# Autodesk Inventor assembly: assembly_support
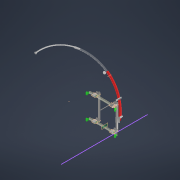
[picture p0: Inventor's stored thumbnail of the model, 180x180]
Saved by Autodesk Inventor 2021 (Build 250183000, 183)
## iProperties
Created: 2021-05-11
Part Number: assembly_support
Document SubType Name: Assembly
Designer: Watchdog
Author: Watchdog
## Documents named in this file (6)
- C:\Users\Watchdog\OneDrive - Flinders\Advn Mech Design Shared\6_Development\2_Design\inventor\support\assembly_support.iam
- C:\Users\Watchdog\OneDrive - Flinders\Advn Mech Design Shared\6_Development\2_Design\inventor\support\roof_bar\ext_roof bar assembly.iam
- C:\Users\Watchdog\OneDrive - Flinders\Advn Mech Design Shared\6_Development\2_Design\inventor\connection\assembly_connector.iam
- C:\Users\Watchdog\OneDrive - Flinders\Advn Mech Design Shared\6_Development\2_Design\inventor\assembly_hoop.iam
- C:\Users\Watchdog\OneDrive - Flinders\Advn Mech Design Shared\6_Development\2_Design\inventor\support\assembly_truss.iam
- C:\Users\Watchdog\OneDrive - Flinders\Advn Mech Design Shared\6_Development\2_Design\inventor\support\support_frame_x.ipt
## Components (9 placed, 5 different names)
1. ext_roof bar assembly:1 [sub-assembly] — Flush:6, Flush:7, Flush:8, Mate:15, Mate:16, Mate:18, Mate:20
2. ext_roof bar assembly:2 [sub-assembly] — Flush:3, Flush:4, Flush:5, Flush:6, Flush:7, Flush:8, Flush:9, Mate:11, Mate:13, Mate:14
3. assembly_connector:1 [sub-assembly] — Flush:9, Mate:11, Mate:21
4. assembly_connector:2 [sub-assembly] — Mate:13, Mate:14, Flush:11, Mate:27
5. assembly_connector:3 [sub-assembly] — Mate:15, Mate:16, Flush:10, Flush:11, Symmetry:1, Mate:26, Mate:28
6. assembly_connector:4 [sub-assembly] — Mate:18, Mate:20, Mate:22, Mate:23, Flush:10, Symmetry:1
7. assembly_hoop:1 [sub-assembly] — Mate:21, Mate:22, Mate:23, Mate:24, Mate:29, Flush:12
8. assembly_truss:1 [sub-assembly] — Mate:24, Mate:29, Flush:12
9. support_frame_x:1 — Mate:26, Mate:27, Mate:28
## Relationships (26: Mate 15, Flush 10, Symmetry 1)
- Flush:3: ext_roof bar assembly:2
- Flush:4: ext_roof bar assembly:2
- Flush:5: ext_roof bar assembly:2
- Flush:6 (900 mm): ext_roof bar assembly:1 ↔ ext_roof bar assembly:2
- Flush:7: ext_roof bar assembly:1 ↔ ext_roof bar assembly:2
- Flush:8: ext_roof bar assembly:1 ↔ ext_roof bar assembly:2
- Flush:9: ext_roof bar assembly:2 ↔ assembly_connector:1
- Mate:11: ext_roof bar assembly:2 ↔ assembly_connector:1
- Mate:13: ext_roof bar assembly:2 ↔ assembly_connector:2
- Mate:14: ext_roof bar assembly:2 ↔ assembly_connector:2
- Mate:15: ext_roof bar assembly:1 ↔ assembly_connector:3
- Mate:16: ext_roof bar assembly:1 ↔ assembly_connector:3
- Mate:18: ext_roof bar assembly:1 ↔ assembly_connector:4
- Mate:20: ext_roof bar assembly:1 ↔ assembly_connector:4
- Mate:21: assembly_connector:1 ↔ assembly_hoop:1
- Mate:22: assembly_connector:4 ↔ assembly_hoop:1
- Mate:23: assembly_connector:4 ↔ assembly_hoop:1
- Mate:24: assembly_hoop:1 ↔ assembly_truss:1
- Flush:10 (-700 mm): assembly_connector:3 ↔ assembly_connector:4
- Flush:11: assembly_connector:2 ↔ assembly_connector:3
- Symmetry:1: assembly_connector:3 ↔ assembly_connector:4
- Mate:26: assembly_connector:3 ↔ support_frame_x:1
- Mate:27: assembly_connector:2 ↔ support_frame_x:1
- Mate:28: assembly_connector:3 ↔ support_frame_x:1
- Mate:29: assembly_hoop:1 ↔ assembly_truss:1
- Flush:12: assembly_hoop:1 ↔ assembly_truss:1
